# Autodesk Inventor assembly: v2-VersaPlanetary-1stage-with-775pro-20161031
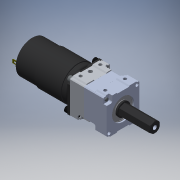
[picture p0: Inventor's stored thumbnail of the model, 180x180]
Saved by Autodesk Inventor 2016 (Build 200138000, 138)
## iProperties
Created: 2016-10-31
Part Number: v2-VersaPlanetary-1stage-with-775pro-20161031
Description: STEP AP214
Document SubType Name: Assembly
Designer: 589013
Sending System: SolidWorks 2016
Preprocessor: SwSTEP 2.0
Title: 217-4973_1stage_775pro.STEP
Revision Number: ANY
## Documents named in this file (17)
- C:\Users\smiku\GrabCAD\Power Hawks CAD\VEXpro Resources\Gearboxes\Versaplanetary Gearbox with 775 Pro\v2-VersaPlanetary-1stage-with-775pro-20161031.iam
- C:\Users\smiku\GrabCAD\Power Hawks CAD\VEXpro Resources\Gearboxes\Versaplanetary Gearbox with 775 Pro\217-2625-026 Rev1.ipt
- C:\Users\smiku\GrabCAD\Power Hawks CAD\VEXpro Resources\Gearboxes\Versaplanetary Gearbox with 775 Pro\217-2742-001 Rev4.ipt
- C:\Users\smiku\GrabCAD\Power Hawks CAD\VEXpro Resources\Gearboxes\Versaplanetary Gearbox with 775 Pro\217-2625-017 Rev1_9714K61.ipt
- C:\Users\smiku\GrabCAD\Power Hawks CAD\VEXpro Resources\Gearboxes\Versaplanetary Gearbox with 775 Pro\217-2625-003 Rev1.ipt
- C:\Users\smiku\GrabCAD\Power Hawks CAD\VEXpro Resources\Gearboxes\Versaplanetary Gearbox with 775 Pro\217-2625-018 Rev1_98541A410.ipt
- C:\Users\smiku\GrabCAD\Power Hawks CAD\VEXpro Resources\Gearboxes\Versaplanetary Gearbox with 775 Pro\832-1750-Ring-Gear-Screw_SSA0832-0500ZC.ipt
- C:\Users\smiku\GrabCAD\Power Hawks CAD\VEXpro Resources\Gearboxes\Versaplanetary Gearbox with 775 Pro\217-2625-025 Rev1.ipt
- C:\Users\smiku\GrabCAD\Power Hawks CAD\VEXpro Resources\Gearboxes\Versaplanetary Gearbox with 775 Pro\217-4649-002 Rev1_SSA0832-0500ZC.ipt
- C:\Users\smiku\GrabCAD\Power Hawks CAD\VEXpro Resources\Gearboxes\Versaplanetary Gearbox with 775 Pro\217-4649-006 Rev1_SSA0004-008BA.ipt
- C:\Users\smiku\GrabCAD\Power Hawks CAD\VEXpro Resources\Gearboxes\Versaplanetary Gearbox with 775 Pro\217-2822-002 Rev4.ipt
- C:\Users\smiku\GrabCAD\Power Hawks CAD\VEXpro Resources\Gearboxes\Versaplanetary Gearbox with 775 Pro\217-4347-000 Rev1.ipt
- C:\Users\smiku\GrabCAD\Power Hawks CAD\VEXpro Resources\Gearboxes\Versaplanetary Gearbox with 775 Pro\217-2820 Rev1_Public.iam
- C:\Users\smiku\GrabCAD\Power Hawks CAD\VEXpro Resources\Gearboxes\Versaplanetary Gearbox with 775 Pro\217-2816-001 Rev1.ipt
- C:\Users\smiku\GrabCAD\Power Hawks CAD\VEXpro Resources\Gearboxes\Versaplanetary Gearbox with 775 Pro\217-4649-001 Rev1.ipt
- C:\Users\smiku\GrabCAD\Power Hawks CAD\VEXpro Resources\Gearboxes\Versaplanetary Gearbox with 775 Pro\217-4649-007 Rev1_94105A824.ipt
- C:\Users\smiku\GrabCAD\Power Hawks CAD\VEXpro Resources\Gearboxes\Versaplanetary Gearbox with 775 Pro\217-2625-013 Rev2.ipt
## Components (20 placed, 20 different names)
1. 217-2625-026 Rev1_1
2. 217-2742-001 Rev4_2
3. 217-2742-001 Rev4_3 — Insert:1
4. 217-2625-017 Rev1_9714K61_4
5. 217-2625-003 Rev1_5 — Insert:1
6. 217-2625-018 Rev1_98541A410_6
7. 832-1750-Ring-Gear-Screw_SSA0832-0500ZC_7
8. 832-1750-Ring-Gear-Screw_SSA0832-0500ZC_8
9. 217-2625-025 Rev1_9
10. 217-4649-002 Rev1_SSA0832-0500ZC_10
11. 217-4649-002 Rev1_SSA0832-0500ZC_11
12. 217-4649-006 Rev1_SSA0004-008BA_12
13. 217-4649-006 Rev1_SSA0004-008BA_13
14. 217-2822-002 Rev4_14
15. 217-4347-000 Rev1_15
16. 217-2820 Rev1_Public_16 [sub-assembly]
17. 217-2816-001 Rev1_17
18. 217-4649-001 Rev1_18
19. 217-4649-007 Rev1_94105A824_19
20. 217-2625-013 Rev2_20
## Relationships (1: Insert 1)
- Insert:1: 217-2742-001 Rev4_3 ↔ 217-2625-003 Rev1_5
